# Autodesk Inventor assembly: Assembly
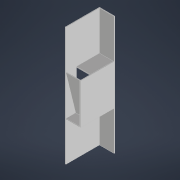
[picture p0: Inventor's stored thumbnail of the model, 180x180]
Saved by Autodesk Inventor 2021.4 (Build 254397000, 397)
## iProperties
Created: 2022-02-22
Part Number: Assembly
Document SubType Name: Assembly
Designer: valen
Author: valen
## Documents named in this file (8)
- D:\Repos\SmartSoccerTableCAD\Parts\goalStructure\Assembly.iam
- D:\Repos\SmartSoccerTableCAD\Parts\goalStructure\TorraumFront.ipt
- D:\Repos\SmartSoccerTableCAD\Parts\goalStructure\TorraumSeiteBalleinwurf.ipt
- D:\Repos\SmartSoccerTableCAD\Parts\goalStructure\TorraumSeitenplatte.ipt
- D:\Repos\SmartSoccerTableCAD\Parts\goalStructure\TorraumSchrägeUntenNEU.ipt
- D:\Repos\SmartSoccerTableCAD\Parts\goalStructure\TorraumSchrägeObenNEU.ipt
- D:\Repos\SmartSoccerTableCAD\Parts\goalStructure\TorraumDecke.ipt
- D:\Repos\SmartSoccerTableCAD\Parts\goalStructure\TorraumHinten.ipt
## Components (7 placed, 7 different names)
1. TorraumFront:1 — Passend:1, Passend:2, Passend:3, Passend:4, Passend:5, Passend:6, Passend:16, Passend:17, Passend:18, Passend:19
2. TorraumSeiteBalleinwurf:1 — Passend:1, Passend:2, Passend:3, Passend:22
3. TorraumSeitenplatte:1 — Passend:4, Passend:5, Passend:6, Passend:20, Passend:21
4. TorraumSchrägeUntenNEU:1
5. TorraumDecke:1 — Passend:16, Passend:17, Passend:18, Passend:23
6. TorraumSchrägeObenNEU:1 — Passend:19, Passend:20
7. TorraumHinten:1 — Passend:21, Passend:22, Passend:23
## Relationships (14: Mate 14)
- Passend:1 [Mate]: TorraumFront:1 ↔ TorraumSeiteBalleinwurf:1
- Passend:2 [Mate]: TorraumFront:1 ↔ TorraumSeiteBalleinwurf:1
- Passend:3 [Mate]: TorraumFront:1 ↔ TorraumSeiteBalleinwurf:1
- Passend:4 [Mate]: TorraumFront:1 ↔ TorraumSeitenplatte:1
- Passend:5 [Mate]: TorraumFront:1 ↔ TorraumSeitenplatte:1
- Passend:6 [Mate]: TorraumFront:1 ↔ TorraumSeitenplatte:1
- Passend:16 [Mate]: TorraumFront:1 ↔ TorraumDecke:1
- Passend:17 [Mate]: TorraumFront:1 ↔ TorraumDecke:1
- Passend:18 [Mate]: TorraumFront:1 ↔ TorraumDecke:1
- Passend:19 [Mate]: TorraumFront:1 ↔ TorraumSchrägeObenNEU:1
- Passend:20 [Mate]: TorraumSeitenplatte:1 ↔ TorraumSchrägeObenNEU:1
- Passend:21 [Mate]: TorraumSeitenplatte:1 ↔ TorraumHinten:1
- Passend:22 [Mate]: TorraumSeiteBalleinwurf:1 ↔ TorraumHinten:1
- Passend:23 [Mate]: TorraumDecke:1 ↔ TorraumHinten:1
